# Autodesk Inventor assembly: Cover Optical Camera Only
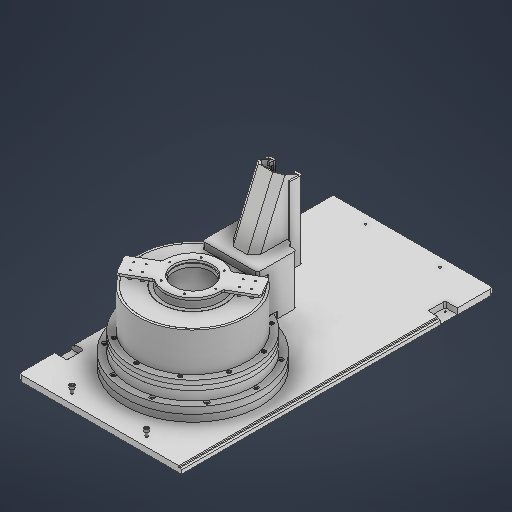
[picture p0: Inventor's stored thumbnail of the model, 512x512]
Saved by Autodesk Inventor 2025 (Build 290162000, 162)
## iProperties
Created: 2025-02-04
Part Number: Cover Optical Camera Only
Document SubType Name: Assembly
Designer: mayhe
Author: mayhe
## Documents named in this file (30)
- C:\Users\mayhe\OneDrive\Documents\GitHub\In-situ-monitoring-of-powder-bed-fusion-additive-manufacturing\system_development\Mithril\v0.2\Model\Cover Optical Camera Only.iam
- C:\Users\mayhe\OneDrive\Documents\GitHub\In-situ-monitoring-of-powder-bed-fusion-additive-manufacturing\system_development\Mithril\v0.2\Model\Cover (Optical Camera).ipt
- C:\Users\mayhe\OneDrive\Documents\GitHub\In-situ-monitoring-of-powder-bed-fusion-additive-manufacturing\system_development\Mithril\v0.2\Model\300mm Housing 1.ipt
- C:\Users\mayhe\OneDrive\Documents\GitHub\In-situ-monitoring-of-powder-bed-fusion-additive-manufacturing\system_development\Mithril\v0.2\Model\Cylinder Spacer Optical Camera.ipt
- C:\Users\mayhe\OneDrive\Documents\GitHub\In-situ-monitoring-of-powder-bed-fusion-additive-manufacturing\system_development\Mithril\v0.2\Model\Cylinder Segment\Cylinder Slidey Bit Housings\Cylinder Slidey Bit Housing Camera only v0.2.ipt
- C:\Users\mayhe\OneDrive\Documents\GitHub\In-situ-monitoring-of-powder-bed-fusion-additive-manufacturing\system_development\Mithril\v0.2\Model\300mm housing 2 Camera.ipt
- C:\Users\mayhe\OneDrive\Documents\GitHub\In-situ-monitoring-of-powder-bed-fusion-additive-manufacturing\system_development\Mithril\v0.2\Model\Cylinder Segment\Cylinder Segment Camera Only\C .Replace - Face.ipt
- C:\Users\mayhe\OneDrive\Documents\GitHub\In-situ-monitoring-of-powder-bed-fusion-additive-manufacturing\system_development\Mithril\v0.2\Model\Cylinder Segment\Cylinder Segment Camera Only.ipt
- C:\Users\mayhe\OneDrive\Documents\GitHub\In-situ-monitoring-of-powder-bed-fusion-additive-manufacturing\system_development\Mithril\v0.2\Model\Cylinder Segment\Cylinder Segment Camera Only\C .Replace - 10.ipt
- C:\Users\mayhe\OneDrive\Documents\GitHub\In-situ-monitoring-of-powder-bed-fusion-additive-manufacturing\system_development\Mithril\v0.2\Model\Cylinder Segment\Cylinder Segment  Camera only v0.2.ipt
- C:\Users\mayhe\OneDrive\Documents\GitHub\In-situ-monitoring-of-powder-bed-fusion-additive-manufacturing\system_development\Mithril\v0.2\Model\Cylinder Segment Holder.ipt
- C:\Users\mayhe\OneDrive\Documents\GitHub\In-situ-monitoring-of-powder-bed-fusion-additive-manufacturing\system_development\Mithril\v0.2\Model\Camera Bracket.ipt
- C:\Users\mayhe\OneDrive\Documents\GitHub\In-situ-monitoring-of-powder-bed-fusion-additive-manufacturing\system_development\Mithril\v0.2\Model\flircamera+lens.ipt
- C:\Users\mayhe\OneDrive\Documents\GitHub\In-situ-monitoring-of-powder-bed-fusion-additive-manufacturing\system_development\Mithril\v0.2\Model\Welding Glass.ipt
- C:\Users\mayhe\OneDrive\Documents\GitHub\In-situ-monitoring-of-powder-bed-fusion-additive-manufacturing\system_development\Mithril\v0.2\Model\Cover^2.ipt
- C:\Users\mayhe\OneDrive\Documents\GitHub\In-situ-monitoring-of-powder-bed-fusion-additive-manufacturing\system_development\Mithril\v0.2\Model\cover^3.ipt
- C:\Users\mayhe\OneDrive\Documents\Inventor\Content Center Files\R2025\en-US\AS 1420\AS 1420 - 1973 - M5 x 20.ipt
- C:\Users\mayhe\OneDrive\Documents\Inventor\Content Center Files\R2025\en-US\ANSI B18.3.1M(1)\ANSI B18.3.1M - M5x0.8 x 50(2).ipt
- C:\Users\mayhe\OneDrive\Documents\Inventor\Content Center Files\R2025\en-US\AS 1420\AS 1420 - 1973 - M5 x 16.ipt
- C:\Users\mayhe\OneDrive\Documents\Inventor\Content Center Files\R2025\en-US\AS 1474(1)\AS 1474 - M5(1).ipt
- C:\Users\mayhe\OneDrive\Documents\GitHub\In-situ-monitoring-of-powder-bed-fusion-additive-manufacturing\system_development\Mithril\v0.2\Model\Head Thing (metal).ipt
- C:\Users\mayhe\OneDrive\Documents\Inventor\Content Center Files\R2025\en-US\AS 1420\AS 1420 - 1973 - M4 x 12.ipt
- C:\Users\mayhe\OneDrive\Documents\Inventor\Content Center Files\R2025\en-US\AS 1420\AS 1420 - 1973 - M3 x 16.ipt
- C:\Users\mayhe\OneDrive\Documents\Inventor\Content Center Files\R2025\en-US\ANSI B18.3.1M(1)\ANSI B18.3.1M - M3x0.5 x 8(2).ipt
- C:\Users\mayhe\OneDrive\Documents\Inventor\Content Center Files\R2025\en-US\ANSI B18.3.1M(1)\ANSI B18.3.1M - M3x0.5 x 35(2).ipt
- C:\Users\mayhe\OneDrive\Documents\Inventor\Content Center Files\R2025\en-US\ANSI B18.3.1M(1)\ANSI B18.3.1M - M3x0.5 x 25(2).ipt
- C:\Users\mayhe\OneDrive\Documents\Inventor\Content Center Files\R2025\en-US\AS 1474(1)\AS 1474 - M3(1).ipt
- C:\Users\mayhe\OneDrive\Documents\Inventor\Content Center Files\R2025\en-US\AS 1420\AS 1420 - 1973 - M4 x 14.ipt
- C:\Users\mayhe\OneDrive\Documents\Inventor\Content Center Files\R2025\en-US\AS 1474(1)\AS 1474 - M4(1).ipt
- C:\Users\mayhe\OneDrive\Documents\Inventor\Content Center Files\R2025\en-US\AS 1420\AS 1420 - 1973 - M6 x 10.ipt
## Components (96 placed, 28 different names)
1. Cover (Optical Camera):1 — Rotational:5, Mate:55, Mate:57
2. 300mm Housing 1:1 — Rotational:5, Rotational:11, Insert:21, Insert:22, Insert:23, Insert:24, Insert:25, Insert:26, Insert:27, Insert:28, Insert:29, Insert:30, Mate:13, Insert:31, Insert:32, Insert:33, Insert:34, Insert:35, Insert:36, Insert:37, Insert:38, Insert:39, Insert:40
3. 300mm housing 2 Camera:2 — Rotational:11, Rotational:12, Insert:1, Insert:2, Insert:3, Insert:4, Insert:5, Insert:6, Insert:7, Insert:8, Insert:9, Insert:10, Insert:41, Insert:42, Insert:43, Insert:44, Insert:45, Insert:46, Insert:47, Insert:48, Insert:49, Insert:50
4. Cylinder Spacer Optical Camera:1 — Rotational:12, Rotational:13
5. Cylinder Segment  Camera only v0.2:1 — Rotational:13, Rotational:14, Rotational:15, Mate:10, Rotational:24, Mate:46, Mate:48
6. Cylinder Slidey Bit Housing Camera only v0.2:1 — Rotational:14, Rotational:18, Flush:2, Mate:11, Insert:11, Insert:12, Insert:13, Insert:14, Insert:15, Insert:17, Insert:18, Insert:19, Insert:20
7. C .Replace - Face:1 — Rotational:16, Rotational:23, Mate:15, Mate:17, Mate:19, Mate:21, Mate:23, Mate:25, Mate:27, Mate:29, Mate:31, Mate:33, Mate:35, Mate:37, Mate:39, Mate:41
8. C .Replace - 10:2 — Rotational:15, Rotational:16
9. Camera Bracket:1 — Rotational:18, Rotational:21, Mate:8, Mate:9, Flush:1, Insert:51, Insert:52, Insert:56, Insert:57, Insert:58, Insert:61, Insert:62, Insert:63
10. flircamera+lens:1 — Rotational:21
11. Welding Glass:1 — Mate:8, Mate:9, Flush:1
12. Cover^2:1 — Mate:10, Flush:2, Mate:11, Rotational:22
13. cover^3:1 — Rotational:22
14. Cylinder Segment Holder:1 — Rotational:24, Insert:64, Insert:65
15. Head Thing (metal):1 — Rotational:23, Mate:14, Mate:16, Mate:18, Mate:20, Mate:22, Mate:24, Mate:26, Mate:28, Mate:30, Mate:32, Mate:34, Mate:36, Mate:38, Mate:40
16. AS 1420 - Metric M6 x 10:3 — Mate:55
17. AS 1420 - Metric M6 x 10:4 — Mate:57
18. AS 1420 - Metric M4 x 14:2 — Insert:65, Mate:47
19. AS 1420 - Metric M4 x 14:1 — Insert:64, Mate:45
20. Broached Socket Head Cap Screw - Metric M3x0.5 x 35:1 — Insert:61, Mate:44
21. Broached Socket Head Cap Screw - Metric M3x0.5 x 35:2 — Insert:62, Mate:43
22. Broached Socket Head Cap Screw - Metric M3x0.5 x 25:1 — Insert:63, Mate:42
23. AS 1420 - Metric M3 x 16:2 — Insert:52
24. AS 1420 - Metric M3 x 16:1 — Insert:51
25. Broached Socket Head Cap Screw - Metric M3x0.5 x 8:1 — Insert:56
26. Broached Socket Head Cap Screw - Metric M3x0.5 x 8:2 — Insert:57
27. Broached Socket Head Cap Screw - Metric M3x0.5 x 8:3 — Insert:58
28. AS 1420 - Metric M5 x 20:1 — Insert:1
29. AS 1420 - Metric M5 x 20:2 — Insert:2
30. AS 1420 - Metric M5 x 20:3 — Insert:3
31. AS 1420 - Metric M5 x 20:4 — Insert:4
32. AS 1420 - Metric M5 x 20:5 — Insert:5
33. AS 1420 - Metric M5 x 20:6 — Insert:6, Mate:12
34. AS 1420 - Metric M5 x 20:7 — Insert:7
35. AS 1420 - Metric M5 x 20:8 — Insert:8
36. AS 1420 - Metric M5 x 20:9 — Insert:9
37. AS 1420 - Metric M5 x 20:10 — Insert:10
38. Broached Socket Head Cap Screw - Metric M5x0.8 x 50:1 — Insert:11
39. Broached Socket Head Cap Screw - Metric M5x0.8 x 50:2 — Insert:12
40. Broached Socket Head Cap Screw - Metric M5x0.8 x 50:3 — Insert:13
41. AS 1420 - Metric M4 x 12:1 — Mate:14, Mate:15
42. AS 1420 - Metric M4 x 12:2 — Mate:16, Mate:17
43. AS 1420 - Metric M4 x 12:3 — Mate:18, Mate:19
44. AS 1420 - Metric M4 x 12:4 — Mate:20, Mate:21
45. AS 1420 - Metric M4 x 12:5 — Mate:22, Mate:23
46. AS 1420 - Metric M4 x 12:6 — Mate:24, Mate:25
47. AS 1420 - Metric M4 x 12:7 — Mate:26, Mate:27
48. AS 1420 - Metric M4 x 12:8 — Mate:28, Mate:29
49. AS 1420 - Metric M4 x 12:9 — Mate:30, Mate:31
50. AS 1420 - Metric M4 x 12:10 — Mate:32, Mate:33
51. AS 1420 - Metric M4 x 12:11 — Mate:34, Mate:35
52. AS 1420 - Metric M4 x 12:12 — Mate:36, Mate:37
53. AS 1420 - Metric M4 x 12:13 — Mate:38, Mate:39
54. AS 1420 - Metric M4 x 12:14 — Mate:40, Mate:41
55. Broached Socket Head Cap Screw - Metric M5x0.8 x 50:4 — Insert:14
56. Broached Socket Head Cap Screw - Metric M5x0.8 x 50:5 — Insert:15
57. Broached Socket Head Cap Screw - Metric M5x0.8 x 50:7 — Insert:17
58. Broached Socket Head Cap Screw - Metric M5x0.8 x 50:8 — Insert:18
59. Broached Socket Head Cap Screw - Metric M5x0.8 x 50:9 — Insert:19
60. Broached Socket Head Cap Screw - Metric M5x0.8 x 50:10 — Insert:20
61. AS 1420 - Metric M5 x 16:1 — Insert:21
62. AS 1420 - Metric M5 x 16:2 — Insert:22
63. AS 1420 - Metric M5 x 16:3 — Insert:23
64. AS 1420 - Metric M5 x 16:4 — Insert:24
65. AS 1420 - Metric M5 x 16:5 — Insert:25
66. AS 1420 - Metric M5 x 16:6 — Insert:26
67. AS 1420 - Metric M5 x 16:7 — Insert:27
68. AS 1420 - Metric M5 x 16:8 — Insert:28
69. AS 1420 - Metric M5 x 16:9 — Insert:29
70. AS 1420 - Metric M5 x 16:10 — Insert:30
71. AS 1474 - Metric M4:2 — Mate:47, Mate:48
72. AS 1474 - Metric M4:1 — Mate:45, Mate:46
73. AS 1474 - Metric M3:1 — Mate:42
74. AS 1474 - Metric M3:2 — Mate:43
75. AS 1474 - Metric M3:3 — Mate:44
76. AS 1474 - Metric M5:13 — Insert:41
77. AS 1474 - Metric M5:14 — Insert:42
78. AS 1474 - Metric M5:15 — Insert:43
79. AS 1474 - Metric M5:16 — Insert:44
80. AS 1474 - Metric M5:17 — Insert:45
81. AS 1474 - Metric M5:18 — Insert:46
82. AS 1474 - Metric M5:19 — Insert:47
83. AS 1474 - Metric M5:20 — Insert:48
84. AS 1474 - Metric M5:21 — Insert:49
85. AS 1474 - Metric M5:22 — Insert:50
86. AS 1474 - Metric M5:1 — Mate:12, Mate:13
87. AS 1474 - Metric M5:3 — Insert:31
88. AS 1474 - Metric M5:4 — Insert:32
89. AS 1474 - Metric M5:5 — Insert:33
90. AS 1474 - Metric M5:6 — Insert:34
91. AS 1474 - Metric M5:7 — Insert:35
92. AS 1474 - Metric M5:8 — Insert:36
93. AS 1474 - Metric M5:9 — Insert:37
94. AS 1474 - Metric M5:10 — Insert:38
95. AS 1474 - Metric M5:11 — Insert:39
96. AS 1474 - Metric M5:12 — Insert:40
## Relationships (117: Insert 59, Mate 43, RevoluteJoint 12, Flush 3)
- Rotational:5 [RevoluteJoint]: Cover (Optical Camera):1 ↔ 300mm Housing 1:1
- Rotational:11 [RevoluteJoint]: 300mm Housing 1:1 ↔ 300mm housing 2 Camera:2
- Rotational:12 [RevoluteJoint]: 300mm housing 2 Camera:2 ↔ Cylinder Spacer Optical Camera:1
- Rotational:13 [RevoluteJoint]: Cylinder Spacer Optical Camera:1 ↔ Cylinder Segment  Camera only v0.2:1
- Rotational:14 [RevoluteJoint]: Cylinder Segment  Camera only v0.2:1 ↔ Cylinder Slidey Bit Housing Camera only v0.2:1
- Rotational:15 [RevoluteJoint]: Cylinder Segment  Camera only v0.2:1 ↔ C .Replace - 10:2
- Rotational:16 [RevoluteJoint]: C .Replace - Face:1 ↔ C .Replace - 10:2
- Rotational:18 [RevoluteJoint]: Cylinder Slidey Bit Housing Camera only v0.2:1 ↔ Camera Bracket:1
- Rotational:21 [RevoluteJoint]: Camera Bracket:1 ↔ flircamera+lens:1
- Mate:8 (0.25 mm): Camera Bracket:1 ↔ Welding Glass:1
- Mate:9: Camera Bracket:1 ↔ Welding Glass:1
- Flush:1 (-30 mm): Camera Bracket:1 ↔ Welding Glass:1
- Mate:10: Cylinder Segment  Camera only v0.2:1 ↔ Cover^2:1
- Flush:2: Cylinder Slidey Bit Housing Camera only v0.2:1 ↔ Cover^2:1
- Mate:11 (2 mm): Cylinder Slidey Bit Housing Camera only v0.2:1 ↔ Cover^2:1
- Rotational:22 [RevoluteJoint]: Cover^2:1 ↔ cover^3:1
- Insert:1: 300mm housing 2 Camera:2 ↔ AS 1420 - Metric M5 x 20:1
- Insert:2: 300mm housing 2 Camera:2 ↔ AS 1420 - Metric M5 x 20:2
- Insert:3: 300mm housing 2 Camera:2 ↔ AS 1420 - Metric M5 x 20:3
- Insert:4: 300mm housing 2 Camera:2 ↔ AS 1420 - Metric M5 x 20:4
- Insert:5: 300mm housing 2 Camera:2 ↔ AS 1420 - Metric M5 x 20:5
- Insert:6: 300mm housing 2 Camera:2 ↔ AS 1420 - Metric M5 x 20:6
- Insert:7: 300mm housing 2 Camera:2 ↔ AS 1420 - Metric M5 x 20:7
- Insert:8: 300mm housing 2 Camera:2 ↔ AS 1420 - Metric M5 x 20:8
- Insert:9: 300mm housing 2 Camera:2 ↔ AS 1420 - Metric M5 x 20:9
- Insert:10: 300mm housing 2 Camera:2 ↔ AS 1420 - Metric M5 x 20:10
- Insert:11: Cylinder Slidey Bit Housing Camera only v0.2:1 ↔ Broached Socket Head Cap Screw - Metric M5x0.8 x 50:1
- Insert:12: Cylinder Slidey Bit Housing Camera only v0.2:1 ↔ Broached Socket Head Cap Screw - Metric M5x0.8 x 50:2
- Insert:13: Cylinder Slidey Bit Housing Camera only v0.2:1 ↔ Broached Socket Head Cap Screw - Metric M5x0.8 x 50:3
- Insert:14: Cylinder Slidey Bit Housing Camera only v0.2:1 ↔ Broached Socket Head Cap Screw - Metric M5x0.8 x 50:4
- Insert:15: Cylinder Slidey Bit Housing Camera only v0.2:1 ↔ Broached Socket Head Cap Screw - Metric M5x0.8 x 50:5
- Insert:17: Cylinder Slidey Bit Housing Camera only v0.2:1 ↔ Broached Socket Head Cap Screw - Metric M5x0.8 x 50:7
- Insert:18: Cylinder Slidey Bit Housing Camera only v0.2:1 ↔ Broached Socket Head Cap Screw - Metric M5x0.8 x 50:8
- Insert:19: Cylinder Slidey Bit Housing Camera only v0.2:1 ↔ Broached Socket Head Cap Screw - Metric M5x0.8 x 50:9
- Insert:20: Cylinder Slidey Bit Housing Camera only v0.2:1 ↔ Broached Socket Head Cap Screw - Metric M5x0.8 x 50:10
- Insert:21: 300mm Housing 1:1 ↔ AS 1420 - Metric M5 x 16:1
- Insert:22: 300mm Housing 1:1 ↔ AS 1420 - Metric M5 x 16:2
- Insert:23: 300mm Housing 1:1 ↔ AS 1420 - Metric M5 x 16:3
- Insert:24: 300mm Housing 1:1 ↔ AS 1420 - Metric M5 x 16:4
- Insert:25: 300mm Housing 1:1 ↔ AS 1420 - Metric M5 x 16:5
- Insert:26: 300mm Housing 1:1 ↔ AS 1420 - Metric M5 x 16:6
- Insert:27: 300mm Housing 1:1 ↔ AS 1420 - Metric M5 x 16:7
- Insert:28: 300mm Housing 1:1 ↔ AS 1420 - Metric M5 x 16:8
- Insert:29: 300mm Housing 1:1 ↔ AS 1420 - Metric M5 x 16:9
- Insert:30: 300mm Housing 1:1 ↔ AS 1420 - Metric M5 x 16:10
- Mate:12: AS 1420 - Metric M5 x 20:6 ↔ AS 1474 - Metric M5:1
- Mate:13: 300mm Housing 1:1 ↔ AS 1474 - Metric M5:1
- Insert:31: 300mm Housing 1:1 ↔ AS 1474 - Metric M5:3
- Insert:32: 300mm Housing 1:1 ↔ AS 1474 - Metric M5:4
- Insert:33: 300mm Housing 1:1 ↔ AS 1474 - Metric M5:5
- Insert:34: 300mm Housing 1:1 ↔ AS 1474 - Metric M5:6
- Insert:35: 300mm Housing 1:1 ↔ AS 1474 - Metric M5:7
- Insert:36: 300mm Housing 1:1 ↔ AS 1474 - Metric M5:8
- Insert:37: 300mm Housing 1:1 ↔ AS 1474 - Metric M5:9
- Insert:38: 300mm Housing 1:1 ↔ AS 1474 - Metric M5:10
- Insert:39: 300mm Housing 1:1 ↔ AS 1474 - Metric M5:11
- Insert:40: 300mm Housing 1:1 ↔ AS 1474 - Metric M5:12
- Insert:41: 300mm housing 2 Camera:2 ↔ AS 1474 - Metric M5:13
- Insert:42: 300mm housing 2 Camera:2 ↔ AS 1474 - Metric M5:14
- Insert:43: 300mm housing 2 Camera:2 ↔ AS 1474 - Metric M5:15
- Insert:44: 300mm housing 2 Camera:2 ↔ AS 1474 - Metric M5:16
- Insert:45: 300mm housing 2 Camera:2 ↔ AS 1474 - Metric M5:17
- Insert:46: 300mm housing 2 Camera:2 ↔ AS 1474 - Metric M5:18
- Insert:47: 300mm housing 2 Camera:2 ↔ AS 1474 - Metric M5:19
- Insert:48: 300mm housing 2 Camera:2 ↔ AS 1474 - Metric M5:20
- Insert:49: 300mm housing 2 Camera:2 ↔ AS 1474 - Metric M5:21
- Insert:50: 300mm housing 2 Camera:2 ↔ AS 1474 - Metric M5:22
- Rotational:23 [RevoluteJoint]: C .Replace - Face:1 ↔ Head Thing (metal):1
- Mate:14: Head Thing (metal):1 ↔ AS 1420 - Metric M4 x 12:1
- Mate:15: C .Replace - Face:1 ↔ AS 1420 - Metric M4 x 12:1
- Mate:16: Head Thing (metal):1 ↔ AS 1420 - Metric M4 x 12:2
- Mate:17: C .Replace - Face:1 ↔ AS 1420 - Metric M4 x 12:2
- Mate:18: Head Thing (metal):1 ↔ AS 1420 - Metric M4 x 12:3
- Mate:19: C .Replace - Face:1 ↔ AS 1420 - Metric M4 x 12:3
- Mate:20: Head Thing (metal):1 ↔ AS 1420 - Metric M4 x 12:4
- Mate:21: C .Replace - Face:1 ↔ AS 1420 - Metric M4 x 12:4
- Mate:22: Head Thing (metal):1 ↔ AS 1420 - Metric M4 x 12:5
- Mate:23: C .Replace - Face:1 ↔ AS 1420 - Metric M4 x 12:5
- Mate:24: Head Thing (metal):1 ↔ AS 1420 - Metric M4 x 12:6
- Mate:25: C .Replace - Face:1 ↔ AS 1420 - Metric M4 x 12:6
- Mate:26: Head Thing (metal):1 ↔ AS 1420 - Metric M4 x 12:7
- Mate:27: C .Replace - Face:1 ↔ AS 1420 - Metric M4 x 12:7
- Mate:28: Head Thing (metal):1 ↔ AS 1420 - Metric M4 x 12:8
- Mate:29: C .Replace - Face:1 ↔ AS 1420 - Metric M4 x 12:8
- Mate:30: Head Thing (metal):1 ↔ AS 1420 - Metric M4 x 12:9
- Mate:31: C .Replace - Face:1 ↔ AS 1420 - Metric M4 x 12:9
- Mate:32: Head Thing (metal):1 ↔ AS 1420 - Metric M4 x 12:10
- Mate:33: C .Replace - Face:1 ↔ AS 1420 - Metric M4 x 12:10
- Mate:34: Head Thing (metal):1 ↔ AS 1420 - Metric M4 x 12:11
- Mate:35: C .Replace - Face:1 ↔ AS 1420 - Metric M4 x 12:11
- Mate:36: Head Thing (metal):1 ↔ AS 1420 - Metric M4 x 12:12
- Mate:37: C .Replace - Face:1 ↔ AS 1420 - Metric M4 x 12:12
- Mate:38: Head Thing (metal):1 ↔ AS 1420 - Metric M4 x 12:13
- Mate:39: C .Replace - Face:1 ↔ AS 1420 - Metric M4 x 12:13
- Mate:40: Head Thing (metal):1 ↔ AS 1420 - Metric M4 x 12:14
- Mate:41: C .Replace - Face:1 ↔ AS 1420 - Metric M4 x 12:14
- Insert:51: Camera Bracket:1 ↔ AS 1420 - Metric M3 x 16:1
- Insert:52: Camera Bracket:1 ↔ AS 1420 - Metric M3 x 16:2
- Insert:56: Camera Bracket:1 ↔ Broached Socket Head Cap Screw - Metric M3x0.5 x 8:1
- Insert:57: Camera Bracket:1 ↔ Broached Socket Head Cap Screw - Metric M3x0.5 x 8:2
- Insert:58: Camera Bracket:1 ↔ Broached Socket Head Cap Screw - Metric M3x0.5 x 8:3
- Insert:61: Camera Bracket:1 ↔ Broached Socket Head Cap Screw - Metric M3x0.5 x 35:1
- Insert:62: Camera Bracket:1 ↔ Broached Socket Head Cap Screw - Metric M3x0.5 x 35:2
- Insert:63: Camera Bracket:1 ↔ Broached Socket Head Cap Screw - Metric M3x0.5 x 25:1
- Mate:42: Broached Socket Head Cap Screw - Metric M3x0.5 x 25:1 ↔ AS 1474 - Metric M3:1
- Mate:43: Broached Socket Head Cap Screw - Metric M3x0.5 x 35:2 ↔ AS 1474 - Metric M3:2
- Mate:44: Broached Socket Head Cap Screw - Metric M3x0.5 x 35:1 ↔ AS 1474 - Metric M3:3
- Rotational:24 [RevoluteJoint]: Cylinder Segment  Camera only v0.2:1 ↔ Cylinder Segment Holder:1
- Insert:64: Cylinder Segment Holder:1 ↔ AS 1420 - Metric M4 x 14:1
- Insert:65: Cylinder Segment Holder:1 ↔ AS 1420 - Metric M4 x 14:2
- Mate:45: AS 1420 - Metric M4 x 14:1 ↔ AS 1474 - Metric M4:1
- Mate:46: Cylinder Segment  Camera only v0.2:1 ↔ AS 1474 - Metric M4:1
- Mate:47: AS 1420 - Metric M4 x 14:2 ↔ AS 1474 - Metric M4:2
- Mate:48: Cylinder Segment  Camera only v0.2:1 ↔ AS 1474 - Metric M4:2
- Flush:3 (128.5875 mm)
- Mate:55: Cover (Optical Camera):1 ↔ AS 1420 - Metric M6 x 10:3
- Mate:57: Cover (Optical Camera):1 ↔ AS 1420 - Metric M6 x 10:4
